# Autodesk Inventor assembly: Ensamble V3
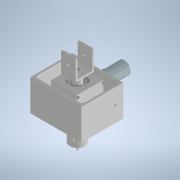
[picture p0: Inventor's stored thumbnail of the model, 180x180]
Saved by Autodesk Inventor 2020.3 (Build 243373000, 373)
## iProperties
Created: 2021-02-09
Part Number: Ensamble V3
Document SubType Name: Assembly
Designer: Yu Jinyu
Author: Yu Jinyu
## Documents named in this file (17)
- C:\Users\Yu Jinyu\OneDrive\Escritorio\Yaw Roll Nuevo\Ensamble V3.iam
- C:\Users\Yu Jinyu\OneDrive\Escritorio\Diseno\Rodamiento\Design Accelerator\Bearing2.iam
- C:\Users\Yu Jinyu\OneDrive\Escritorio\Diseno\soporte 2.0.ipt
- C:\Users\Yu Jinyu\OneDrive\Escritorio\Yaw Roll Nuevo\Motor Banebot.iam
- C:\Users\Yu Jinyu\OneDrive\Escritorio\Yaw Roll Nuevo\brazo conexion.iam
- C:\Users\Yu Jinyu\OneDrive\Documentos\Inventor\Content Center Files\R2020\en-US\AS 1111\AS 1111 - M5 x 25.ipt
- C:\Users\Yu Jinyu\OneDrive\Documentos\Inventor\Content Center Files\R2020\en-US\AS 1110\AS 1110 - M5 x 16.ipt
- C:\Users\Yu Jinyu\OneDrive\Escritorio\Yaw Roll Nuevo\hub polulu.ipt
- C:\Users\Yu Jinyu\OneDrive\Documentos\Inventor\Content Center Files\R2020\en-US\AS 1110\AS 1110 - M3 x 10.ipt
- C:\Users\Yu Jinyu\OneDrive\Escritorio\Yaw Roll Nuevo\Pololu37D.ipt
- C:\Users\Yu Jinyu\OneDrive\Documentos\Inventor\Content Center Files\R2020\en-US\AS 1421(1)\AS 1421 - M3x10 Cone Point.ipt
- C:\Users\Yu Jinyu\OneDrive\Documentos\Inventor\Content Center Files\R2020\en-US\AS 1421(1)\AS 1421 - M3x5 Cone Point.ipt
- C:\Users\Yu Jinyu\OneDrive\Escritorio\Yaw Roll Nuevo\tapa.ipt
- C:\Users\Yu Jinyu\OneDrive\Documentos\Inventor\Content Center Files\R2020\en-US\AS 1110\AS 1110 - M3 x 6.ipt
- C:\Users\Yu Jinyu\OneDrive\Escritorio\Yaw Roll Nuevo\eje escalonado V2.ipt
- C:\Users\Yu Jinyu\OneDrive\Escritorio\Yaw Roll Nuevo\caja conexion.ipt
- C:\Users\Yu Jinyu\OneDrive\Escritorio\Yaw Roll Nuevo\Ensamble V3\Design Accelerator\Bearing3.iam
## Components (39 placed, 15 different names)
1. Bearing:1 [sub-assembly] — Insert:1, Insert:2, Insert:3
2. soporte 2.0:1 — Insert:1, Insert:16, Insert:17, Insert:18, Insert:20, Insert:21, Insert:22, Insert:23, Insert:32
3. Motor Banebot:1 [sub-assembly] — Insert:2
4. brazo conexion:1 [sub-assembly] — Insert:3, Insert:4
5. AS 1111 - Metric M5 x 25:1 — Insert:4
6. AS 1110 - Metric M5 x 16:4
7. AS 1110 - Metric M5 x 16:3
8. AS 1110 - Metric M5 x 16:2
9. AS 1110 - Metric M5 x 16:1
10. hub polulu:2 — Insert:15, Rigid:1, Rigid:2, Rigid:3, Rigid:4, Insert:22
11. AS 1110 - Metric M3 x 10:1 — Insert:21
12. AS 1110 - Metric M3 x 10:2 — Insert:18
13. AS 1110 - Metric M3 x 10:3 — Insert:17
14. AS 1110 - Metric M3 x 10:4 — Insert:20
15. AS 1110 - Metric M3 x 10:5
16. AS 1110 - Metric M3 x 10:6 — Insert:16
17. Pololu37D:1 — Insert:15
18. AS 1421 Cone Point - Metric M3x10 Cone Point:1 — Rigid:1
19. AS 1421 Cone Point - Metric M3x10 Cone Point:2 — Rigid:2
20. AS 1421 Cone Point - Metric M3x5 Cone Point:3 — Rigid:3
21. AS 1421 Cone Point - Metric M3x5 Cone Point:7 — Rigid:4
22. tapa:2 — Insert:23, Insert:24, Insert:25, Insert:26, Insert:27, Insert:28, Insert:29, Insert:30, Insert:31
23. AS 1110 - Metric M3 x 6:1 — Insert:24
24. AS 1110 - Metric M3 x 6:2 — Insert:25
25. AS 1110 - Metric M3 x 6:3 — Insert:26
26. AS 1110 - Metric M3 x 6:4 — Insert:27
27. AS 1110 - Metric M5 x 16:5 — Insert:28
28. AS 1110 - Metric M5 x 16:6 — Insert:29
29. AS 1110 - Metric M5 x 16:7 — Insert:30
30. AS 1110 - Metric M5 x 16:8 — Insert:31
31. eje escalonado V2:1 — Insert:32, Insert:40
32. caja conexion:1 — Insert:34, Insert:35, Insert:36, Insert:37, Insert:38, Insert:39
33. AS 1110 - Metric M3 x 10:7 — Insert:34
34. AS 1110 - Metric M3 x 10:8 — Insert:35
35. AS 1110 - Metric M3 x 10:9 — Insert:36
36. AS 1110 - Metric M3 x 10:10 — Insert:37
37. AS 1110 - Metric M3 x 10:11 — Insert:38
38. AS 1110 - Metric M3 x 10:12 — Insert:39
39. Bearing:3 [sub-assembly] — Insert:40
## Relationships (32: Insert 28, WeldJoint 4)
- Insert:1: Bearing:1 ↔ soporte 2.0:1
- Insert:2: Bearing:1 ↔ Motor Banebot:1
- Insert:3 (-14.288 mm): Bearing:1 ↔ brazo conexion:1
- Insert:4: brazo conexion:1 ↔ AS 1111 - Metric M5 x 25:1
- Insert:15: hub polulu:2 ↔ Pololu37D:1
- Rigid:1 [WeldJoint]: hub polulu:2 ↔ AS 1421 Cone Point - Metric M3x10 Cone Point:1
- Rigid:2 [WeldJoint]: hub polulu:2 ↔ AS 1421 Cone Point - Metric M3x10 Cone Point:2
- Rigid:3 [WeldJoint]: hub polulu:2 ↔ AS 1421 Cone Point - Metric M3x5 Cone Point:3
- Rigid:4 [WeldJoint]: hub polulu:2 ↔ AS 1421 Cone Point - Metric M3x5 Cone Point:7
- Insert:16: soporte 2.0:1 ↔ AS 1110 - Metric M3 x 10:6
- Insert:17: soporte 2.0:1 ↔ AS 1110 - Metric M3 x 10:3
- Insert:18: soporte 2.0:1 ↔ AS 1110 - Metric M3 x 10:2
- Insert:20: soporte 2.0:1 ↔ AS 1110 - Metric M3 x 10:4
- Insert:21: soporte 2.0:1 ↔ AS 1110 - Metric M3 x 10:1
- Insert:22: soporte 2.0:1 ↔ hub polulu:2
- Insert:23: soporte 2.0:1 ↔ tapa:2
- Insert:24: tapa:2 ↔ AS 1110 - Metric M3 x 6:1
- Insert:25: tapa:2 ↔ AS 1110 - Metric M3 x 6:2
- Insert:26: tapa:2 ↔ AS 1110 - Metric M3 x 6:3
- Insert:27: tapa:2 ↔ AS 1110 - Metric M3 x 6:4
- Insert:28: tapa:2 ↔ AS 1110 - Metric M5 x 16:5
- Insert:29: tapa:2 ↔ AS 1110 - Metric M5 x 16:6
- Insert:30: tapa:2 ↔ AS 1110 - Metric M5 x 16:7
- Insert:31: tapa:2 ↔ AS 1110 - Metric M5 x 16:8
- Insert:32: soporte 2.0:1 ↔ eje escalonado V2:1
- Insert:34: caja conexion:1 ↔ AS 1110 - Metric M3 x 10:7
- Insert:35: caja conexion:1 ↔ AS 1110 - Metric M3 x 10:8
- Insert:36: caja conexion:1 ↔ AS 1110 - Metric M3 x 10:9
- Insert:37: caja conexion:1 ↔ AS 1110 - Metric M3 x 10:10
- Insert:38: caja conexion:1 ↔ AS 1110 - Metric M3 x 10:11
- Insert:39: caja conexion:1 ↔ AS 1110 - Metric M3 x 10:12
- Insert:40: eje escalonado V2:1 ↔ Bearing:3
